# Autodesk Inventor assembly: ASY MSC D-ring
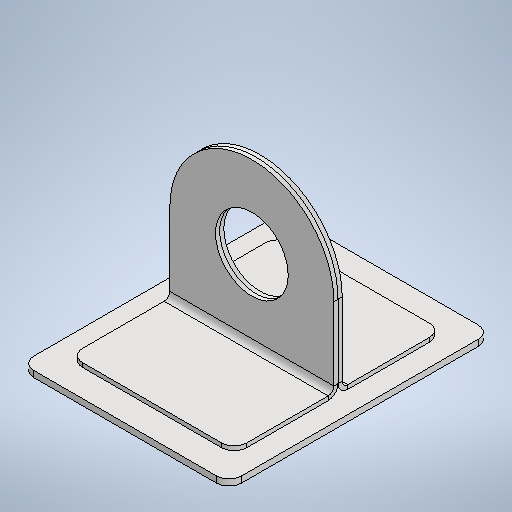
[picture p0: Inventor's stored thumbnail of the model, 512x512]
Saved by Autodesk Inventor 2025 (Build 290162010, 162A)
## iProperties
Created: 2024-11-20
Part Number: ASY MSC D-ring
Document SubType Name: Assembly
Designer: admin
Author: admin
## Documents named in this file (3)
- C:\Users\admin\YandexDisk-badmisterfox\домашниий пк\Inventor\Manturovo\Manturovo_Se-clar\ASY MSC D-ring.iam
- C:\Users\admin\YandexDisk-badmisterfox\домашниий пк\Inventor\Manturovo\Manturovo_Se-clar\D-ring 11.ipt
- C:\Users\admin\YandexDisk-badmisterfox\домашниий пк\Inventor\Manturovo\Manturovo_Se-clar\MSC 820 D-ring plate.ipt
## Components (3 placed, 2 different names)
1. D-ring 11:1
2. D-ring 11:2 — Mate:1, Mate:2, Mate:3
3. Part1:1 — Mate:1, Mate:4, Mate:5, Mate:6
## Relationships (7: Mate 6, WeldJoint 1)
- [WeldJoint]: D-ring 11:1 ↔ D-ring 11:2
- Mate:1: D-ring 11:2 ↔ Part1:1
- Mate:2: D-ring 11:2
- Mate:3: D-ring 11:2
- Mate:4: Part1:1
- Mate:5: Part1:1
- Mate:6: Part1:1
